# Autodesk Inventor assembly: CL3-100
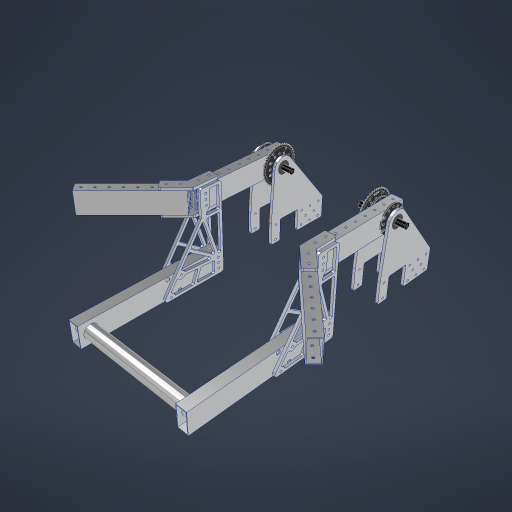
[picture p0: Inventor's stored thumbnail of the model, 512x512]
Saved by Autodesk Inventor 2023.4 (Build 274418000, 418)
## iProperties
Created: 2025-01-28
Part Number: CL3-100
Document SubType Name: Assembly
Designer: slick
Mass: 5966.39 g
Surface Area: 14199.1 cm^2
Volume: 2256.64 cm^3
Density: 2.64392 g/cm^3
Author: slick
## Documents named in this file (18)
- C:\Users\brand\OneDrive\Documents\GitHub\robotics 23\2025-ReefScape---CAD\Climber\CL3\CL3-100.iam
- C:\Users\brand\OneDrive\Documents\GitHub\robotics 23\2025-ReefScape---CAD\Climber\CL3\CL3-001.ipt
- C:\Users\brand\OneDrive\Documents\GitHub\robotics 23\2025-ReefScape---CAD\Climber\CL3\CL3-002.ipt
- C:\Users\brand\OneDrive\Documents\GitHub\robotics 23\2025-ReefScape---CAD\Climber\CL3\CL3-003.ipt
- C:\Users\brand\OneDrive\Documents\GitHub\robotics 23\2025-ReefScape---CAD\Climber\CL3\CL3-004.ipt
- C:\Users\brand\OneDrive\Documents\GitHub\robotics 23\2025-ReefScape---CAD\Climber\CL3\CL3-006.ipt
- C:\Users\brand\OneDrive\Documents\GitHub\robotics 23\2025-ReefScape---CAD\Field Items\Full Field\FE-2025\GE-25201.iam
- C:\Users\brand\OneDrive\Documents\GitHub\robotics 23\2025-ReefScape---CAD\Climber\CL3\CL3-007.ipt
- C:\Users\brand\OneDrive\Documents\GitHub\robotics 23\2025-ReefScape---CAD\Climber\CL3\CL3-009.ipt
- C:\Users\brand\OneDrive\Documents\GitHub\robotics 23\2025-ReefScape---CAD\Elevator\EL2\EL2-005.ipt
- C:\Users\brand\OneDrive\Documents\GitHub\robotics 23\2025-ReefScape---CAD\Climber\CL3\CL3-010.ipt
- C:\Users\brand\OneDrive\Documents\GitHub\robotics 23\2025-ReefScape---CAD\Climber\CL3\CL3-011.ipt
- C:\Users\brand\OneDrive\Documents\GitHub\robotics 23\2025-ReefScape---CAD\COMMON PARTS\BEARINGS\0_500_Hex_ID_x_1_125_OD_x_0_313_WD_Flanged_Bearing_v2_217-3875.ipt
- C:\Users\brand\OneDrive\Documents\GitHub\robotics 23\2025-ReefScape---CAD\COMMON PARTS\Z - STEPS\WCP-1388\WCP-1388.ipt
- C:\Users\brand\OneDrive\Documents\GitHub\robotics 23\2025-ReefScape---CAD\COMMON PARTS\SPROCKETS\25\WCP-0967 42t 25_chain.ipt
- C:\Users\brand\OneDrive\Documents\GitHub\robotics 23\2025-ReefScape---CAD\Climber\CL3\CL3-012.ipt
- C:\Users\brand\OneDrive\Documents\GitHub\robotics 23\2025-ReefScape---CAD\Climber\CL3\CL3-013.ipt
- C:\Users\brand\OneDrive\Documents\GitHub\robotics 23\2025-ReefScape---CAD\Climber\CL3\CL3-014.ipt
## Components (48 placed, 17 different names)
1. CL3-001:1 — Flush:24, Insert:5, Insert:6, Insert:7, Insert:11, Insert:12, Insert:13, Insert:14, Mate:43, Mate:44, Mate:51, Mate:52, Mate:53, Mate:54, Mate:55, Angle:4, Insert:43, Insert:44
2. CL3-002:1 — Flush:24, Insert:3, Insert:4, Insert:8
3. CL3-003:1 — Insert:26, Insert:27, Mate:56, Mate:57, Insert:48, Insert:49, Insert:50, Insert:51
4. CL3-001:2 — Insert:18, Insert:19, Insert:20, Insert:21, Insert:24, Insert:25, Insert:41, Mate:65, Insert:42, Mate:66, Mate:67
5. CL3-002:2 — Insert:22, Insert:23
6. CL3-003:2 — Mate:29, Flush:26, Flush:27, Mate:33, Mate:34, Insert:15, Insert:16, Insert:17, Insert:45, Insert:46, Insert:47
7. CL3-004:3 — Mate:41, Flush:31, Flush:32, Insert:29, Angle:4, Symmetry:2
8. CL3-004:4 — Insert:39, Mate:68, Flush:33, Symmetry:3
9. CL3-006:1 — Tangent:1, Mate:21, Mate:33, Mate:34, Mate:56, Mate:57
10. GE-25201:1 [sub-assembly] — Mate:20, Tangent:1, Mate:21
11. CL3-007:1 — Mate:29, Flush:26, Flush:27
12. CL3-009:1 — Insert:3, Insert:4, Insert:5, Insert:6
13. CL3-009:2 — Insert:7, Insert:8
14. CL3-013:1 — Insert:43, Insert:44
15. CL3-010:1 — Insert:11, Insert:12, Flush:29
16. CL3-010:2 — Insert:13, Insert:14, Insert:16, Insert:17
17. EL2-005:3 — Insert:15, Insert:45
18. CL3-009:3 — Insert:18, Insert:19
19. CL3-009:4 — Insert:20, Insert:21, Insert:22, Insert:23
20. CL3-010:3 — Insert:25, Flush:29, Flush:30
21. CL3-010:4 — Insert:24, Insert:26, Insert:27, Flush:30
22. CL3-011:1 — Mate:42, Mate:55
23. CL3-004:5 — Mate:41, Flush:31, Flush:32, Insert:28, Symmetry:2, Flush:34, Flush:35
24. 0_500_Hex_ID_x_1_125_OD_x_0_313_WD_Flanged_Bearing_v2_217-3875:1 — Insert:28, Mate:42
25. 0_500_Hex_ID_x_1_125_OD_x_0_313_WD_Flanged_Bearing_v2_217-3875:2 — Insert:29
26. WCP-1388:1 — Mate:43, Mate:44, Mate:49, Mate:50, Mate:51, Mate:58
27. WCP-1388:2 — Mate:52, Mate:53, Mate:54, Symmetry:1
28. WCP-0967 42t 25_chain:1 — Mate:49, Mate:50, Insert:30, Insert:31, Insert:32, Insert:33, Symmetry:1
29. CL3-012:1 — Insert:30, Mate:58
30. CL3-012:2 — Insert:31
31. CL3-012:3 — Insert:33
32. CL3-012:4 — Insert:32
33. CL3-004:6 — Insert:40, Mate:68, Flush:33, Flush:34, Flush:35, Symmetry:3
34. CL3-011:2 — Mate:64, Mate:67
35. 0_500_Hex_ID_x_1_125_OD_x_0_313_WD_Flanged_Bearing_v2_217-3875:3 — Insert:39
36. 0_500_Hex_ID_x_1_125_OD_x_0_313_WD_Flanged_Bearing_v2_217-3875:4 — Insert:40, Mate:64
37. WCP-1388:3 — Insert:41, Mate:65
38. WCP-1388:4 — Insert:42, Mate:66, Symmetry:4
39. WCP-0967 42t 25_chain:2 — Symmetry:4
40. CL3-012:5
41. CL3-012:6
42. CL3-012:7
43. CL3-012:8
44. CL3-014:1 — Insert:46
45. CL3-014:2 — Insert:47
46. CL3-014:3 — Insert:50
47. CL3-014:4 — Insert:51
48. EL2-005:4 — Insert:48, Insert:49
## Relationships (92: Insert 46, Mate 30, Flush 10, Symmetry 4, Tangent 1, Angle 1)
- Mate:20: GE-25201:1
- Tangent:1: CL3-006:1 ↔ GE-25201:1
- Mate:21 (-76.2 mm): CL3-006:1 ↔ GE-25201:1
- Flush:24: CL3-001:1 ↔ CL3-002:1
- Mate:29: CL3-003:2 ↔ CL3-007:1
- Flush:26: CL3-003:2 ↔ CL3-007:1
- Flush:27: CL3-003:2 ↔ CL3-007:1
- Insert:3: CL3-002:1 ↔ CL3-009:1
- Insert:4: CL3-002:1 ↔ CL3-009:1
- Insert:5: CL3-001:1 ↔ CL3-009:1
- Insert:6: CL3-001:1 ↔ CL3-009:1
- Insert:7: CL3-001:1 ↔ CL3-009:2
- Insert:8: CL3-002:1 ↔ CL3-009:2
- Mate:33: CL3-003:2 ↔ CL3-006:1
- Mate:34: CL3-003:2 ↔ CL3-006:1
- Insert:11: CL3-001:1 ↔ CL3-010:1
- Insert:12: CL3-001:1 ↔ CL3-010:1
- Insert:13: CL3-001:1 ↔ CL3-010:2
- Insert:14: CL3-001:1 ↔ CL3-010:2
- Insert:15: CL3-003:2 ↔ EL2-005:3
- Insert:16: CL3-003:2 ↔ CL3-010:2
- Insert:17: CL3-003:2 ↔ CL3-010:2
- Insert:18: CL3-001:2 ↔ CL3-009:3
- Insert:19: CL3-001:2 ↔ CL3-009:3
- Insert:20: CL3-001:2 ↔ CL3-009:4
- Insert:21: CL3-001:2 ↔ CL3-009:4
- Insert:22: CL3-002:2 ↔ CL3-009:4
- Insert:23: CL3-002:2 ↔ CL3-009:4
- Insert:24: CL3-001:2 ↔ CL3-010:4
- Insert:25: CL3-001:2 ↔ CL3-010:3
- Flush:29: CL3-010:1 ↔ CL3-010:3
- Insert:26: CL3-003:1 ↔ CL3-010:4
- Insert:27: CL3-003:1 ↔ CL3-010:4
- Flush:30: CL3-010:3 ↔ CL3-010:4
- Mate:41 (50.8 mm): CL3-004:3 ↔ CL3-004:5
- Flush:31: CL3-004:3 ↔ CL3-004:5
- Flush:32: CL3-004:3 ↔ CL3-004:5
- Insert:28: CL3-004:5 ↔ 0_500_Hex_ID_x_1_125_OD_x_0_313_WD_Flanged_Bearing_v2_217-3875:1
- Insert:29: CL3-004:3 ↔ 0_500_Hex_ID_x_1_125_OD_x_0_313_WD_Flanged_Bearing_v2_217-3875:2
- Mate:42: CL3-011:1 ↔ 0_500_Hex_ID_x_1_125_OD_x_0_313_WD_Flanged_Bearing_v2_217-3875:1
- Mate:43: CL3-001:1 ↔ WCP-1388:1
- Mate:44: CL3-001:1 ↔ WCP-1388:1
- Mate:49: WCP-1388:1 ↔ WCP-0967 42t 25_chain:1
- Mate:50: WCP-1388:1 ↔ WCP-0967 42t 25_chain:1
- Mate:51: CL3-001:1 ↔ WCP-1388:1
- Mate:52: CL3-001:1 ↔ WCP-1388:2
- Mate:53: CL3-001:1 ↔ WCP-1388:2
- Mate:54: CL3-001:1 ↔ WCP-1388:2
- Mate:55: CL3-001:1 ↔ CL3-011:1
- Angle:4 (270 deg): CL3-001:1 ↔ CL3-004:3
- Mate:56: CL3-003:1 ↔ CL3-006:1
- Mate:57: CL3-003:1 ↔ CL3-006:1
- Insert:30: WCP-0967 42t 25_chain:1 ↔ CL3-012:1
- Mate:58: WCP-1388:1 ↔ CL3-012:1
- Insert:31: WCP-0967 42t 25_chain:1 ↔ CL3-012:2
- Insert:32: WCP-0967 42t 25_chain:1 ↔ CL3-012:4
- Insert:33: WCP-0967 42t 25_chain:1 ↔ CL3-012:3
- Symmetry:1: WCP-1388:2 ↔ WCP-0967 42t 25_chain:1
- Symmetry:2: CL3-004:3 ↔ CL3-004:5
- Mate:59
- [Mate]: CL3-011:2 ↔ 0_500_Hex_ID_x_1_125_OD_x_0_313_WD_Flanged_Bearing_v2_217-3875:3
- [Mate]: WCP-1388:3 ↔ WCP-0967 42t 25_chain:2
- [Mate]: WCP-1388:3 ↔ WCP-0967 42t 25_chain:2
- [Insert]: WCP-0967 42t 25_chain:2 ↔ CL3-012:5
- [Mate]: WCP-1388:3 ↔ CL3-012:5
- [Insert]: WCP-0967 42t 25_chain:2 ↔ CL3-012:6
- [Insert]: WCP-0967 42t 25_chain:2 ↔ CL3-012:8
- [Insert]: WCP-0967 42t 25_chain:2 ↔ CL3-012:7
- Insert:39: CL3-004:4 ↔ 0_500_Hex_ID_x_1_125_OD_x_0_313_WD_Flanged_Bearing_v2_217-3875:3
- Insert:40: CL3-004:6 ↔ 0_500_Hex_ID_x_1_125_OD_x_0_313_WD_Flanged_Bearing_v2_217-3875:4
- Mate:64: CL3-011:2 ↔ 0_500_Hex_ID_x_1_125_OD_x_0_313_WD_Flanged_Bearing_v2_217-3875:4
- Insert:41: CL3-001:2 ↔ WCP-1388:3
- Mate:65: CL3-001:2 ↔ WCP-1388:3
- Insert:42: CL3-001:2 ↔ WCP-1388:4
- Mate:66: CL3-001:2 ↔ WCP-1388:4
- Mate:67: CL3-001:2 ↔ CL3-011:2
- Mate:68 (50.8 mm): CL3-004:4 ↔ CL3-004:6
- Flush:33: CL3-004:4 ↔ CL3-004:6
- Flush:34: CL3-004:5 ↔ CL3-004:6
- Flush:35: CL3-004:5 ↔ CL3-004:6
- Symmetry:3: CL3-004:4 ↔ CL3-004:6
- Symmetry:4: WCP-1388:4 ↔ WCP-0967 42t 25_chain:2
- Mate:69
- Insert:43: CL3-001:1 ↔ CL3-013:1
- Insert:44: CL3-001:1 ↔ CL3-013:1
- Insert:45: CL3-003:2 ↔ EL2-005:3
- Insert:46: CL3-003:2 ↔ CL3-014:1
- Insert:47: CL3-003:2 ↔ CL3-014:2
- Insert:48: CL3-003:1 ↔ EL2-005:4
- Insert:49: CL3-003:1 ↔ EL2-005:4
- Insert:50: CL3-003:1 ↔ CL3-014:3
- Insert:51: CL3-003:1 ↔ CL3-014:4
## Named parameters: d209_d182 = 0 mm, d210_d190 = 0 mm, d211_d191 = 0 mm, d212_d202 = 0 mm, d213_d203 = 0 mm, d214_d204 = 0 mm, d215_d205 = 0 mm, d216_d206 = 0 mm
